# Autodesk Inventor assembly: base_link
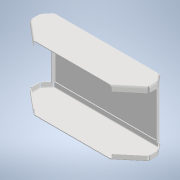
[picture p0: Inventor's stored thumbnail of the model, 180x180]
Saved by Autodesk Inventor 2021 (Build 250183000, 183)
## iProperties
Created: 2021-07-21
Part Number: base_link
Document SubType Name: Weldment
Designer: admin
Weld Material: Welded Aluminum-6061
Author: admin
## Documents named in this file (3)
- C:\Users\admin\OneDrive - Universidad Tecnológica de Panamá\PLATAFORMA_MOVIL_V1.0\DESIGN\DESIGN_PARTS\base_link.iam
- C:\Users\admin\OneDrive - Universidad Tecnológica de Panamá\PLATAFORMA_MOVIL_V1.0\DESIGN\DESIGN_PARTS\Fondo.ipt
- C:\Users\admin\OneDrive - Universidad Tecnológica de Panamá\PLATAFORMA_MOVIL_V1.0\DESIGN\DESIGN_PARTS\Lateral_A.ipt
## Components (3 placed, 2 different names)
1. Fondo:1 — Rígido:1, Rígido:2
2. Lateral_A:1 — Rígido:1
3. Lateral_A:2 — Rígido:2
## Relationships (2: WeldJoint 2)
- Rígido:1 [WeldJoint]: Fondo:1 ↔ Lateral_A:1
- Rígido:2 [WeldJoint]: Fondo:1 ↔ Lateral_A:2
